# Autodesk Inventor assembly: Griber samlet
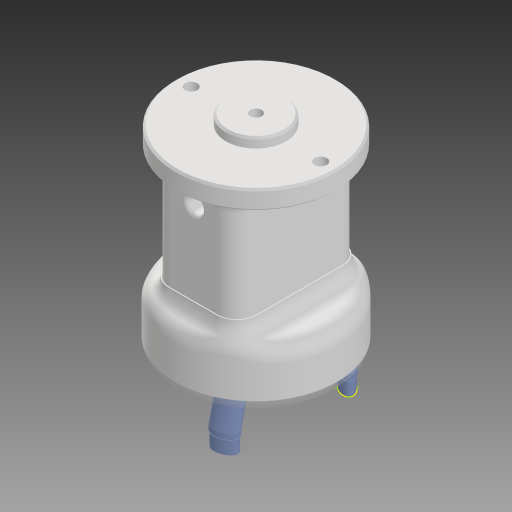
[picture p0: Inventor's stored thumbnail of the model, 512x512]
Saved by Autodesk Inventor 2024 (Build 280153000, 153)
## iProperties
Created: 2024-03-08
Part Number: Griber samlet
Document SubType Name: Assembly
Designer: Faber
Author: Faber
## Documents named in this file (6)
- C:\Users\Bluex\OneDrive - Syddansk Universitet\2. Semester\Semesterprojekt i autonome robotter\Inventor filer\Griber samlet.iam
- C:\Users\Bluex\OneDrive - Syddansk Universitet\2. Semester\Semesterprojekt i autonome robotter\Inventor filer\Sol_Gear.ipt
- C:\Users\Bluex\OneDrive - Syddansk Universitet\2. Semester\Semesterprojekt i autonome robotter\Inventor filer\Gear_Hus.ipt
- C:\Users\Bluex\OneDrive - Syddansk Universitet\2. Semester\Semesterprojekt i autonome robotter\Inventor filer\Gear_Hus_Laag.ipt
- C:\Users\Bluex\OneDrive - Syddansk Universitet\2. Semester\Semesterprojekt i autonome robotter\Inventor filer\Motor_Hus.ipt
- C:\Users\Bluex\Documents\GitHub\Autonome_Robotter\3D_inventor_robor_hånd\Planet_Gear_finger_V2.ipt
## Components (7 placed, 5 different names)
1. Sol_Gear:1 — Mate:2, Mate:3, Rotation:1, Rotation:2, Rotation:3
2. Gear_Hus:1 — Mate:2, Mate:3, Mate:4, Mate:5, Mate:6, Mate:7, Mate:8, Mate:9, Mate:10, Mate:11, Mate:12, Mate:13, Mate:14, Mate:15
3. Gear_Hus_Laag:1 — Mate:4, Mate:5, Mate:6
4. Motor_Hus:1 — Mate:7, Mate:8, Mate:9
5. Planet_Gear_finger_V2:1 — Mate:11, Mate:13, Rotation:3
6. Planet_Gear_finger_V2:2 — Mate:10, Mate:14, Rotation:1
7. Planet_Gear_finger_V2:3 — Mate:12, Mate:15, Rotation:2
## Relationships (17: Mate 14, RelateRotation 3)
- Mate:2: Sol_Gear:1 ↔ Gear_Hus:1
- Mate:3: Sol_Gear:1 ↔ Gear_Hus:1
- Mate:4: Gear_Hus:1 ↔ Gear_Hus_Laag:1
- Mate:5: Gear_Hus:1 ↔ Gear_Hus_Laag:1
- Mate:6: Gear_Hus:1 ↔ Gear_Hus_Laag:1
- Mate:7: Gear_Hus:1 ↔ Motor_Hus:1
- Mate:8: Gear_Hus:1 ↔ Motor_Hus:1
- Mate:9: Gear_Hus:1 ↔ Motor_Hus:1
- Mate:10: Gear_Hus:1 ↔ Planet_Gear_finger_V2:2
- Mate:11: Gear_Hus:1 ↔ Planet_Gear_finger_V2:1
- Mate:12: Gear_Hus:1 ↔ Planet_Gear_finger_V2:3
- Mate:13: Gear_Hus:1 ↔ Planet_Gear_finger_V2:1
- Mate:14: Gear_Hus:1 ↔ Planet_Gear_finger_V2:2
- Mate:15: Gear_Hus:1 ↔ Planet_Gear_finger_V2:3
- Rotation:1 [RelateRotation] (0.3846 ul): Sol_Gear:1 ↔ Planet_Gear_finger_V2:2
- Rotation:2 [RelateRotation] (0.3846 ul): Sol_Gear:1 ↔ Planet_Gear_finger_V2:3
- Rotation:3 [RelateRotation] (0.3846 ul): Sol_Gear:1 ↔ Planet_Gear_finger_V2:1
